# Autodesk Inventor assembly: LightSwitchAssembly
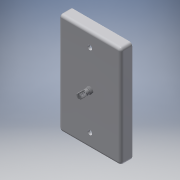
[picture p0: Inventor's stored thumbnail of the model, 180x180]
Saved by Autodesk Inventor 2018 (Build 220112000, 112)
## iProperties
Created: 2018-02-16
Part Number: LightSwitchAssembly
Document SubType Name: Assembly
Designer: brutu
Author: brutu
## Documents named in this file (3)
- C:\Users\brutu\Desktop\LocalGit\seniorproject\hardware\mechanical\LightSwitchAssembly.iam
- C:\Users\brutu\Desktop\LocalGit\seniorproject\hardware\mechanical\LightSwitchCover.ipt
- C:\Users\brutu\Desktop\LocalGit\seniorproject\hardware\mechanical\PEC11-4215F-S24.ipt
## Components (2 placed, 2 different names)
1. LightSwitchCover:1 — Mate:1, Mate:2
2. PEC11-4215F-S24:1 — Mate:1, Mate:2
## Relationships (2: Mate 2)
- Mate:1: LightSwitchCover:1 ↔ PEC11-4215F-S24:1
- Mate:2: LightSwitchCover:1 ↔ PEC11-4215F-S24:1
